# Autodesk Inventor assembly: pinza
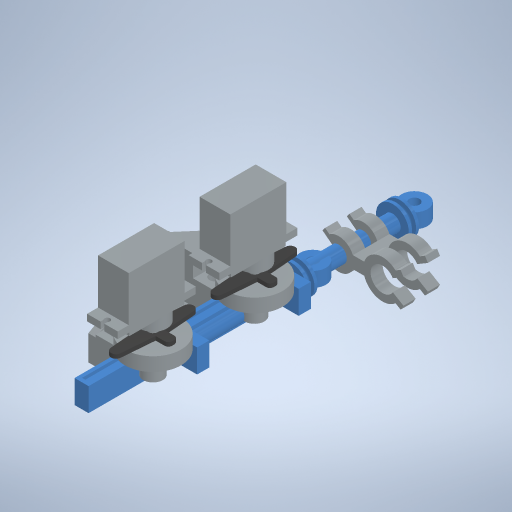
[picture p0: Inventor's stored thumbnail of the model, 512x512]
Saved by Autodesk Inventor 2024.3 (Build 283343000, 343)
## iProperties
Created: 2024-09-30
Part Number: pinza
Description: pinza
Document SubType Name: Assembly
Designer: User
Author: User
## Documents named in this file (8)
- C:\Users\User\Documents\Universidad Octavo Semestre\Robotica Industrial\matlab\SCARA\mariana_scara_final\mariana_scara_final\pinza.iam
- C:\Users\User\Documents\Universidad Octavo Semestre\Robotica Industrial\matlab\SCARA\mariana_scara_final\mariana_scara_final\servomotor.ipt
- C:\Users\User\Documents\Universidad Octavo Semestre\Robotica Industrial\matlab\SCARA\mariana_scara_final\mariana_scara_final\acople_servo.ipt
- C:\Users\User\Documents\Universidad Octavo Semestre\Robotica Industrial\matlab\SCARA\mariana_scara_final\mariana_scara_final\cremallera1.ipt
- C:\Users\User\Documents\Universidad Octavo Semestre\Robotica Industrial\matlab\SCARA\mariana_scara_final\mariana_scara_final\polea_ensayo.ipt
- C:\Users\User\Documents\Universidad Octavo Semestre\Robotica Industrial\matlab\SCARA\mariana_scara_final\mariana_scara_final\lamina-1 - copia.ipt
- C:\Users\User\Documents\Universidad Octavo Semestre\Robotica Industrial\matlab\SCARA\mariana_scara_final\mariana_scara_final\soporte_pinza.ipt
- C:\Users\User\Documents\Universidad Octavo Semestre\Robotica Industrial\matlab\SCARA\mariana_scara_final\mariana_scara_final\union.ipt
## Components (15 placed, 7 different names)
1. servomotor
2. acople_servo
3. cremallera1
4. polea_ensayo
5. lamina-1 - copia
6. lamina-1 - copia:1
7. soporte_pinza
8. acople_servo:1
9. cremallera1:1 — Mate:2
10. lamina-1 - copia:2
11. lamina-1 - copia:3
12. soporte_pinza:1
13. servomotor:1
14. polea_ensayo:1
15. union:1 — Mate:2
## Relationships (1: Mate 1)
- Mate:2: cremallera1:1 ↔ union:1
